# Autodesk Inventor assembly: sm_connection
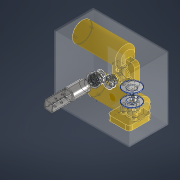
[picture p0: Inventor's stored thumbnail of the model, 180x180]
Saved by Autodesk Inventor 2021 (Build 250183000, 183)
## iProperties
Created: 2021-06-22
Part Number: sm_connection
Document SubType Name: Assembly
Designer: Watchdog
Mass: 4851.98 g
Surface Area: 5151.62 cm^2
Volume: 1601.19 cm^3
Density: 3.03024 g/cm^3
Author: Watchdog
## Documents named in this file (8)
- C:\Users\Watchdog\OneDrive - Flinders\Advn Mech Design Shared\6_Development\2_Design\inventor\securing_mechanism\connection\sm_connection.iam
- C:\Users\Watchdog\OneDrive - Flinders\Advn Mech Design Shared\6_Development\2_Design\inventor\securing_mechanism\connection\gear_khk_SUS1-28J10.ipt
- C:\Users\Watchdog\OneDrive - Flinders\Advn Mech Design Shared\6_Development\2_Design\inventor\securing_mechanism\connection\member_s2c.ipt
- C:\Users\Watchdog\OneDrive - Flinders\Advn Mech Design Shared\6_Development\2_Design\inventor\support\reel\motor.ipt
- C:\Users\Watchdog\OneDrive - Flinders\Advn Mech Design Shared\6_Development\2_Design\inventor\securing_mechanism\connection\box.ipt
- C:\Users\Watchdog\OneDrive - Flinders\Advn Mech Design Shared\6_Development\2_Design\inventor\securing_mechanism\connection\secureingReel.ipt
- C:\Users\Watchdog\OneDrive - Flinders\Advn Mech Design Shared\6_Development\2_Design\inventor\securing_mechanism\connection\bearingSeat.ipt
- C:\Users\Watchdog\OneDrive - Flinders\Advn Mech Design Shared\6_Development\2_Design\inventor\securing_mechanism\connection\SKF_16100.iam
## Components (9 placed, 7 different names)
1. gear_khk_SUS1-28J10:1 — Mate:22, Mate:23
2. member_s2c:1 — Mate:2, Mate:6, Mate:19, Mate:20, Mate:22, Mate:23
3. motor:1 — Angle:3, Mate:10, Mate:25, Angle:5, Flush:2, Mate:26
4. gear_khk_SUS1-28J10:2 — Mate:25, Angle:5, Flush:2
5. motor:2 — Angle:3, Mate:11, Mate:12, Mate:13, Mate:14, Angle:4, Mate:15
6. box:1 — Mate:6, Mate:10, Mate:11, Mate:12, Mate:13, Mate:17, Mate:21, Mate:24, Mate:26, Flush:3, Flush:4
7. secureingReel:1 — Mate:14, Angle:4, Mate:15
8. bearingSeat:1 — Mate:17, Mate:21
9. SKF_16100:1 [sub-assembly] — Mate:19, Mate:20, Mate:24
## Relationships (23: Mate 17, Angle 3, Flush 3)
- Mate:2: member_s2c:1
- Mate:6: member_s2c:1 ↔ box:1
- Angle:3 (0 deg): motor:1 ↔ motor:2
- Mate:10: motor:1 ↔ box:1
- Mate:11: motor:2 ↔ box:1
- Mate:12: motor:2 ↔ box:1
- Mate:13: motor:2 ↔ box:1
- Mate:14: motor:2 ↔ secureingReel:1
- Angle:4 (180 deg): motor:2 ↔ secureingReel:1
- Mate:15: motor:2 ↔ secureingReel:1
- Mate:17: box:1 ↔ bearingSeat:1
- Mate:19: member_s2c:1 ↔ SKF_16100:1
- Mate:20: member_s2c:1 ↔ SKF_16100:1
- Mate:21: box:1 ↔ bearingSeat:1
- Mate:22: gear_khk_SUS1-28J10:1 ↔ member_s2c:1
- Mate:23: gear_khk_SUS1-28J10:1 ↔ member_s2c:1
- Mate:24: box:1 ↔ SKF_16100:1
- Mate:25: motor:1 ↔ gear_khk_SUS1-28J10:2
- Angle:5 (180 deg): motor:1 ↔ gear_khk_SUS1-28J10:2
- Flush:2: motor:1 ↔ gear_khk_SUS1-28J10:2
- Mate:26: motor:1 ↔ box:1
- Flush:3: box:1
- Flush:4: box:1
